# Autodesk Inventor assembly: Übertragung des Zahnriemens
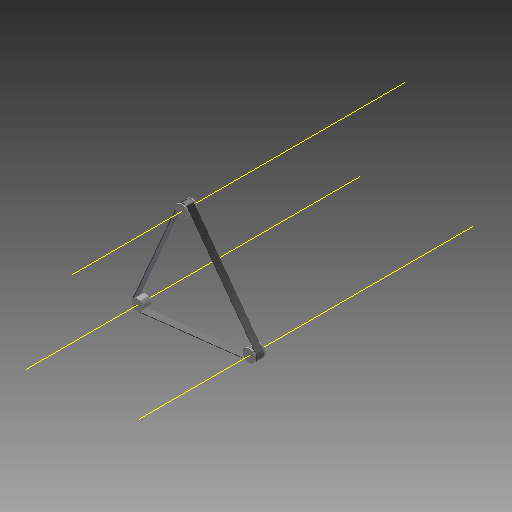
[picture p0: Inventor's stored thumbnail of the model, 512x512]
Saved by Autodesk Inventor 2018.3 (Build 223284000, 284)
## iProperties
Created: 2018-09-15
Part Number: Übertragung des Zahnriemens
Document SubType Name: Assembly
Designer: JochenAlt
ClientObjectVersion: 1
Author: JochenAlt
## Documents named in this file (5)
- D:\Projects\Ondine\CAD\Spindle\LiftGearBeltConstruction\Konstruktions-Assistent\Übertragung des Zahnriemens1.iam
- D:\Projects\Ondine\CAD\Spindle\LiftGearBeltConstruction\Konstruktions-Assistent\Zahnriemen1.ipt
- D:\Projects\Ondine\CAD\Spindle\LiftGearBeltConstruction\Konstruktions-Assistent\Synchrone Riemenscheibe11.ipt
- D:\Projects\Ondine\CAD\Spindle\LiftGearBeltConstruction\Konstruktions-Assistent\Synchrone Riemenscheibe21.ipt
- D:\Projects\Ondine\CAD\Spindle\LiftGearBeltConstruction\Konstruktions-Assistent\Synchrone Riemenscheibe31.ipt
## Components (4 placed, 4 different names)
1. Zahnriemen:1 — Fluchtend:1, Passend:1, Passend:2, Fluchtend:2, Passend:3, Passend:4, Fluchtend:3, Passend:5, Passend:6
2. Synchrone Riemenscheibe1:1 — Fluchtend:1, Passend:1, Passend:2, Drehung:1, Drehung:2
3. Synchrone Riemenscheibe2:1 — Fluchtend:2, Passend:3, Drehung:1, Passend:4
4. Synchrone Riemenscheibe3:1 — Fluchtend:3, Passend:5, Drehung:2, Passend:6
## Relationships (11: Mate 6, Flush 3, RelateRotation 2)
- Fluchtend:1 [Flush]: Zahnriemen:1 ↔ Synchrone Riemenscheibe1:1
- Passend:1 [Mate]: Zahnriemen:1 ↔ Synchrone Riemenscheibe1:1
- Passend:2 [Mate]: Zahnriemen:1 ↔ Synchrone Riemenscheibe1:1
- Fluchtend:2 [Flush]: Zahnriemen:1 ↔ Synchrone Riemenscheibe2:1
- Passend:3 [Mate]: Zahnriemen:1 ↔ Synchrone Riemenscheibe2:1
- Drehung:1 [RelateRotation] (1 ul): Synchrone Riemenscheibe1:1 ↔ Synchrone Riemenscheibe2:1
- Passend:4 [Mate]: Zahnriemen:1 ↔ Synchrone Riemenscheibe2:1
- Fluchtend:3 [Flush]: Zahnriemen:1 ↔ Synchrone Riemenscheibe3:1
- Passend:5 [Mate]: Zahnriemen:1 ↔ Synchrone Riemenscheibe3:1
- Drehung:2 [RelateRotation] (1 ul): Synchrone Riemenscheibe1:1 ↔ Synchrone Riemenscheibe3:1
- Passend:6 [Mate]: Zahnriemen:1 ↔ Synchrone Riemenscheibe3:1
